# Autodesk Inventor assembly: Motor
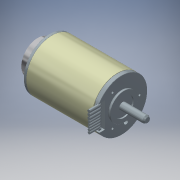
[picture p0: Inventor's stored thumbnail of the model, 180x180]
Saved by Autodesk Inventor 2018.3 (Build 223284000, 284)
## iProperties
Created: 2018-06-30
Part Number: Motor
Material: Generisch
Document SubType Name: Assembly
Designer: JochenAlt
Author: JochenAlt
## Documents named in this file (4)
- D:\Projects\FlowerPot\CAD\Motor.iam
- D:\Projects\FlowerPot\CAD\Maxxon Motor 272766.ipt
- Maxxon Motor 272766.ipt
- D:\Projects\FlowerPot\CAD\Mounting Hub.ipt
## Components (2 placed, 2 different names)
1. Maxxon Motor 272766:1 — Passend:1, Passend:2
2. Mounting Hub:1 — Passend:1, Passend:2
## Relationships (2: Mate 2)
- Passend:1 [Mate]: Maxxon Motor 272766:1 ↔ Mounting Hub:1
- Passend:2 [Mate] (0.5 mm): Maxxon Motor 272766:1 ↔ Mounting Hub:1
